# Autodesk Inventor assembly: Manipulator
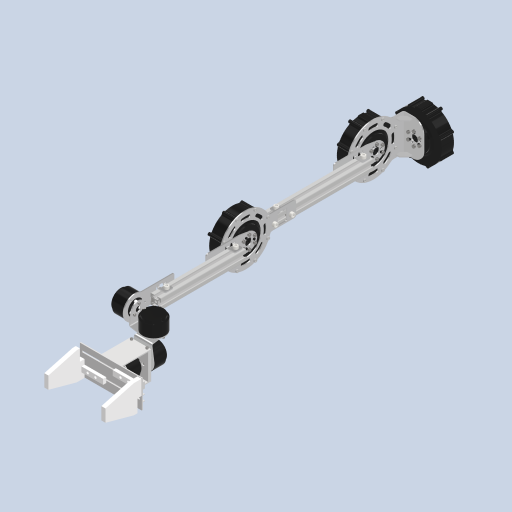
[picture p0: Inventor's stored thumbnail of the model, 512x512]
Saved by Autodesk Inventor 2023 (Build 270158000, 158)
## iProperties
Created: 2024-11-08
Part Number: Manipulator
Document SubType Name: Assembly
Designer: kiyo
Author: kiyo
## Documents named in this file (20)
- D:\GitHub\inventor\syu-si\OfficeRobot\Manipulator\Manipulator.iam
- D:\GitHub\inventor\syu-si\OfficeRobot\ReadyMade\Steadywin\GIM8108-8.iam
- D:\GitHub\inventor\syu-si\OfficeRobot\Manipulator\elbow-pitch-bracket.ipt
- D:\GitHub\inventor\syu-si\OfficeRobot\ReadyMade\Screw\M3_6mm.ipt
- D:\GitHub\inventor\syu-si\OfficeRobot\ReadyMade\Steadywin\GIM3505-8_with-driver.ipt
- D:\GitHub\inventor\syu-si\OfficeRobot\Manipulator\wrist_roll_plate.ipt
- D:\GitHub\inventor\syu-si\OfficeRobot\Manipulator\wrist-pitch-plate.ipt
- D:\GitHub\inventor\syu-si\OfficeRobot\ReadyMade\Screw\M2-5_6mm.ipt
- D:\GitHub\inventor\syu-si\OfficeRobot\ReadyMade\Screw\CBSH3-8.ipt
- D:\GitHub\inventor\syu-si\OfficeRobot\ReadyMade\Screw\FWSJJ-D5-V2_6-T4_5.ipt
- D:\GitHub\inventor\syu-si\OfficeRobot\ReadyMade\Screw\M2-5_10mm.ipt
- D:\GitHub\inventor\syu-si\OfficeRobot\ReadyMade\Screw\HNTU5-5.ipt
- D:\GitHub\inventor\syu-si\OfficeRobot\Manipulator\pitch_plate_20mm.ipt
- D:\GitHub\inventor\syu-si\OfficeRobot\Manipulator\sholder_roll_bracket.ipt
- D:\GitHub\inventor\syu-si\OfficeRobot\ReadyMade\Screw\SCB5-22.ipt
- D:\GitHub\inventor\syu-si\OfficeRobot\ReadyMade\Screw\SCB5-8.ipt
- D:\GitHub\inventor\syu-si\OfficeRobot\Manipulator\Hand_tyokudou.iam
- D:\GitHub\inventor\syu-si\OfficeRobot\Manipulator\wrist-yaw-plate.ipt
- D:\GitHub\inventor\syu-si\OfficeRobot\ReadyMade\Aluminum-frame\NFS5-2020-200-AV10-BV179.ipt
- D:\GitHub\inventor\syu-si\OfficeRobot\ReadyMade\Aluminum-frame\NFS5-2020-165-AV10-BV144.ipt
## Components (91 placed, 19 different names)
1. sholder_roll_bracket:1 — 挿入:350, 挿入:361, 挿入:362, 挿入:363, 挿入:364, 挿入:365, 挿入:366, 挿入:414, 挿入:415
2. wrist-yaw-plate:1 — 挿入:456, 挿入:457, 挿入:458, 挿入:459
3. wrist_roll_plate:2 — 挿入:402, 挿入:403, 挿入:404, 挿入:405, 挿入:406, 挿入:407, 挿入:452
4. Hand_tyokudou:1 [sub-assembly] — 挿入:431, 挿入:434, 挿入:435, 挿入:462, 角度:59, 角度:60
5. pitch_plate_20mm:1 — 挿入:465, 正接:44, メイト:62, 角度:74, 角度:75, 正接:45, メイト:65, メイト:79, 正接:53, 角度:81
6. HNTU5-5:30 — 角度:75
7. SCB5-8:15 — 正接:45, メイト:65
8. elbow-pitch-bracket:1 — 挿入:467, 挿入:468, メイト:81, 正接:55, メイト:85, 正接:57, メイト:87, 正接:58
9. pitch_plate_20mm:2 — 挿入:469, メイト:89, 正接:59, 正接:60, 角度:80, 角度:82
10. wrist-pitch-plate:1 — メイト:70, メイト:71, メイト:72, 正接:46, 正接:47, 正接:48, 正接:49, 角度:76, 角度:77, 角度:78, 正接:50, 正接:51, 挿入:470, 挿入:471
11. NFS5-2020-200-AV10-BV179:1 — 角度:79, メイト:86, メイト:88
12. HNTU5-5:31
13. SCB5-22:9 — メイト:79, 正接:53
14. HNTU5-5:32
15. SCB5-22:10 — メイト:81, 正接:55
16. HNTU5-5:33 — 角度:79, メイト:86
17. SCB5-8:16 — メイト:85, 正接:57
18. HNTU5-5:34 — メイト:88
19. SCB5-8:17 — メイト:87, 正接:58
20. HNTU5-5:35 — 角度:80
21. SCB5-22:11 — メイト:89, 正接:59, 正接:60
22. NFS5-2020-165-AV10-BV144:1
23. M3_6mm:1 — 挿入:337
24. M3_6mm:2 — 挿入:336
25. M3_6mm:3 — 挿入:334
26. M3_6mm:4 — 挿入:338
27. M3_6mm:5 — 挿入:339
28. M3_6mm:6 — 挿入:335
29. M3_6mm:7
30. M3_6mm:8
31. M3_6mm:9
32. M3_6mm:10
33. M3_6mm:11
34. M3_6mm:12
35. M3_6mm:13 — 挿入:361
36. M3_6mm:14 — 挿入:363
37. M3_6mm:15 — 挿入:362
38. M3_6mm:16 — 挿入:364
39. M3_6mm:17 — 挿入:365
40. M3_6mm:18 — 挿入:366
41. CBSH3-8:1 — 挿入:307
42. CBSH3-8:2 — 挿入:308
43. CBSH3-8:3 — 挿入:302
44. CBSH3-8:4 — 挿入:304, 挿入:415
45. CBSH3-8:5 — 挿入:309
46. CBSH3-8:6 — 挿入:303
47. CBSH3-8:7 — 挿入:305
48. CBSH3-8:8 — 挿入:306
49. CBSH3-8:9 — 挿入:332
50. CBSH3-8:10 — 挿入:327, 挿入:468
51. CBSH3-8:11 — 挿入:330
52. CBSH3-8:12 — 挿入:328
53. CBSH3-8:13 — 挿入:329
54. CBSH3-8:14 — 挿入:331
55. CBSH3-8:15 — 挿入:326
56. CBSH3-8:16 — 挿入:333
57. M2-5_6mm:13
58. M2-5_6mm:14
59. M2-5_6mm:15
60. M2-5_10mm:7 — 挿入:402
61. M2-5_10mm:8 — 挿入:403
62. M2-5_10mm:9 — 挿入:404
63. M2-5_10mm:10 — 挿入:430
64. M2-5_10mm:11
65. M2-5_10mm:12
66. M2-5_10mm:13 — 挿入:453, 挿入:456
67. M2-5_10mm:15 — 挿入:454, 挿入:457
68. M2-5_10mm:14 — 挿入:455, 挿入:458
69. FWSJJ-D5-V2_6-T4_5:16 — 挿入:454
70. FWSJJ-D5-V2_6-T4_5:17 — 挿入:453
71. FWSJJ-D5-V2_6-T4_5:18 — 挿入:455
72. FWSJJ-D5-V2_6-T4_5:10 — 挿入:407
73. FWSJJ-D5-V2_6-T4_5:11 — 挿入:405
74. FWSJJ-D5-V2_6-T4_5:12 — 挿入:406
75. FWSJJ-D5-V2_6-T4_5:13 — 挿入:430, 挿入:431
76. FWSJJ-D5-V2_6-T4_5:14 — 挿入:434
77. FWSJJ-D5-V2_6-T4_5:15 — 挿入:435
78. HNTU5-5:22 — 挿入:412, 角度:76
79. SCB5-8:8 — 挿入:412, メイト:72, 正接:49, 正接:50
80. HNTU5-5:23 — 挿入:411, 角度:77
81. SCB5-8:9 — 挿入:411, メイト:71, 正接:48, 正接:51
82. SCB5-22:8 — 挿入:375, メイト:70, 正接:46, 正接:47
83. SCB5-8:7 — 正接:44, メイト:62
84. HNTU5-5:14 — 挿入:375, 角度:78
85. HNTU5-5:21 — 角度:74
86. GIM8108-8:1 [sub-assembly] — 挿入:350, 角度:54, 角度:55, 角度:58
87. GIM8108-8:2 [sub-assembly] — 挿入:302, 挿入:303, 挿入:304, 挿入:305, 挿入:306, 挿入:307, 挿入:308, 挿入:309, 挿入:414, 角度:55, 挿入:465, 角度:81
88. GIM8108-8:3 [sub-assembly] — 挿入:326, 挿入:327, 挿入:328, 挿入:329, 挿入:330, 挿入:331, 挿入:332, 挿入:333, 挿入:334, 挿入:335, 挿入:336, 挿入:337, 挿入:338, 挿入:339, 挿入:467, 挿入:469, 角度:82
89. GIM3505-8_with-driver:9 — 挿入:452, 挿入:470, 挿入:471
90. GIM3505-8_with-driver:8 — 挿入:459
91. GIM3505-8_with-driver:10 — 挿入:462
## Relationships (131: Insert 75, Mate 24, Tangent 18, Angle 14)
- 挿入:302 [Insert] (2 mm): CBSH3-8:3 ↔ GIM8108-8:2
- 挿入:303 [Insert] (2 mm): CBSH3-8:6 ↔ GIM8108-8:2
- 挿入:304 [Insert] (2 mm): CBSH3-8:4 ↔ GIM8108-8:2
- 挿入:305 [Insert] (2 mm): CBSH3-8:7 ↔ GIM8108-8:2
- 挿入:306 [Insert] (2 mm): CBSH3-8:8 ↔ GIM8108-8:2
- 挿入:307 [Insert] (2 mm): CBSH3-8:1 ↔ GIM8108-8:2
- 挿入:308 [Insert] (2 mm): CBSH3-8:2 ↔ GIM8108-8:2
- 挿入:309 [Insert] (2 mm): CBSH3-8:5 ↔ GIM8108-8:2
- 挿入:326 [Insert] (2 mm): CBSH3-8:15 ↔ GIM8108-8:3
- 挿入:327 [Insert] (2 mm): CBSH3-8:10 ↔ GIM8108-8:3
- 挿入:328 [Insert] (2 mm): CBSH3-8:12 ↔ GIM8108-8:3
- 挿入:329 [Insert] (2 mm): CBSH3-8:13 ↔ GIM8108-8:3
- 挿入:330 [Insert] (2 mm): CBSH3-8:11 ↔ GIM8108-8:3
- 挿入:331 [Insert] (2 mm): CBSH3-8:14 ↔ GIM8108-8:3
- 挿入:332 [Insert] (2 mm): CBSH3-8:9 ↔ GIM8108-8:3
- 挿入:333 [Insert] (2 mm): CBSH3-8:16 ↔ GIM8108-8:3
- 挿入:334 [Insert] (2 mm): M3_6mm:3 ↔ GIM8108-8:3
- 挿入:335 [Insert] (2 mm): M3_6mm:6 ↔ GIM8108-8:3
- 挿入:336 [Insert] (2 mm): M3_6mm:2 ↔ GIM8108-8:3
- 挿入:337 [Insert] (2 mm): M3_6mm:1 ↔ GIM8108-8:3
- 挿入:338 [Insert] (2 mm): M3_6mm:4 ↔ GIM8108-8:3
- 挿入:339 [Insert] (2 mm): M3_6mm:5 ↔ GIM8108-8:3
- 挿入:350 [Insert]: sholder_roll_bracket:1 ↔ GIM8108-8:1
- 挿入:361 [Insert]: sholder_roll_bracket:1 ↔ M3_6mm:13
- 挿入:362 [Insert]: sholder_roll_bracket:1 ↔ M3_6mm:15
- 挿入:363 [Insert]: sholder_roll_bracket:1 ↔ M3_6mm:14
- 挿入:364 [Insert]: sholder_roll_bracket:1 ↔ M3_6mm:16
- 挿入:365 [Insert]: sholder_roll_bracket:1 ↔ M3_6mm:17
- 挿入:366 [Insert]: sholder_roll_bracket:1 ↔ M3_6mm:18
- 挿入:375 [Insert] (-0.95 mm): SCB5-22:8 ↔ HNTU5-5:14
- [Insert] (3.2 mm): SCB5-8:7 ↔ HNTU5-5:21
- [Insert]: wrist_roll_plate:2 ↔ M2-5_6mm:13
- [Insert]: wrist_roll_plate:2 ↔ M2-5_6mm:14
- [Insert]: wrist_roll_plate:2 ↔ M2-5_6mm:15
- [Insert]: wrist_roll_plate:2 ↔ GIM3505-8_with-driver:8
- [Insert]: wrist_roll_plate:2 ↔ GIM3505-8_with-driver:8
- 挿入:402 [Insert]: wrist_roll_plate:2 ↔ M2-5_10mm:7
- 挿入:403 [Insert]: wrist_roll_plate:2 ↔ M2-5_10mm:8
- 挿入:404 [Insert]: wrist_roll_plate:2 ↔ M2-5_10mm:9
- 挿入:405 [Insert]: wrist_roll_plate:2 ↔ FWSJJ-D5-V2_6-T4_5:11
- 挿入:406 [Insert]: wrist_roll_plate:2 ↔ FWSJJ-D5-V2_6-T4_5:12
- 挿入:407 [Insert]: wrist_roll_plate:2 ↔ FWSJJ-D5-V2_6-T4_5:10
- 挿入:411 [Insert] (3.5 mm): HNTU5-5:23 ↔ SCB5-8:9
- 挿入:412 [Insert] (3.5 mm): HNTU5-5:22 ↔ SCB5-8:8
- 挿入:414 [Insert]: sholder_roll_bracket:1 ↔ GIM8108-8:2
- 挿入:415 [Insert]: sholder_roll_bracket:1 ↔ CBSH3-8:4
- 挿入:430 [Insert] (2 mm): M2-5_10mm:10 ↔ FWSJJ-D5-V2_6-T4_5:13
- 挿入:431 [Insert]: Hand_tyokudou:1 ↔ FWSJJ-D5-V2_6-T4_5:13
- [Insert] (2 mm): M2-5_10mm:11 ↔ FWSJJ-D5-V2_6-T4_5:14
- [Insert] (2 mm): M2-5_10mm:12 ↔ FWSJJ-D5-V2_6-T4_5:15
- 挿入:434 [Insert]: Hand_tyokudou:1 ↔ FWSJJ-D5-V2_6-T4_5:14
- 挿入:435 [Insert]: Hand_tyokudou:1 ↔ FWSJJ-D5-V2_6-T4_5:15
- 挿入:452 [Insert] (4.5 mm): wrist_roll_plate:2 ↔ GIM3505-8_with-driver:9
- 挿入:453 [Insert] (2 mm): M2-5_10mm:13 ↔ FWSJJ-D5-V2_6-T4_5:17
- 挿入:454 [Insert] (2 mm): M2-5_10mm:15 ↔ FWSJJ-D5-V2_6-T4_5:16
- 挿入:455 [Insert] (2 mm): M2-5_10mm:14 ↔ FWSJJ-D5-V2_6-T4_5:18
- 挿入:456 [Insert]: wrist-yaw-plate:1 ↔ M2-5_10mm:13
- 挿入:457 [Insert]: wrist-yaw-plate:1 ↔ M2-5_10mm:15
- 挿入:458 [Insert]: wrist-yaw-plate:1 ↔ M2-5_10mm:14
- 挿入:459 [Insert] (4.5 mm): wrist-yaw-plate:1 ↔ GIM3505-8_with-driver:8
- [Insert]: wrist-yaw-plate:1 ↔ GIM3505-8_with-driver:10
- [Insert]: wrist-yaw-plate:1 ↔ GIM3505-8_with-driver:10
- 挿入:462 [Insert] (4.5 mm): Hand_tyokudou:1 ↔ GIM3505-8_with-driver:10
- 角度:54 [Angle] (0 deg): GIM8108-8:1
- 角度:55 [Angle] (180 deg): GIM8108-8:1 ↔ GIM8108-8:2
- 角度:58 [Angle] (180 deg): GIM8108-8:1
- 角度:59 [Angle] (0 deg): Hand_tyokudou:1
- 角度:60 [Angle] (0 deg): Hand_tyokudou:1
- 挿入:465 [Insert]: pitch_plate_20mm:1 ↔ GIM8108-8:2
- 正接:44 [Tangent] (0.25 mm): pitch_plate_20mm:1 ↔ SCB5-8:7
- メイト:62 [Mate]: pitch_plate_20mm:1 ↔ SCB5-8:7
- 角度:74 [Angle] (0 deg): pitch_plate_20mm:1 ↔ HNTU5-5:21
- [Insert] (3.2 mm): HNTU5-5:30 ↔ SCB5-8:15
- 角度:75 [Angle] (0 deg): pitch_plate_20mm:1 ↔ HNTU5-5:30
- 正接:45 [Tangent] (0.25 mm): pitch_plate_20mm:1 ↔ SCB5-8:15
- メイト:65 [Mate]: pitch_plate_20mm:1 ↔ SCB5-8:15
- 挿入:467 [Insert]: elbow-pitch-bracket:1 ↔ GIM8108-8:3
- 挿入:468 [Insert]: elbow-pitch-bracket:1 ↔ CBSH3-8:10
- 挿入:469 [Insert]: pitch_plate_20mm:2 ↔ GIM8108-8:3
- メイト:70 [Mate]: wrist-pitch-plate:1 ↔ SCB5-22:8
- メイト:71 [Mate]: wrist-pitch-plate:1 ↔ SCB5-8:9
- メイト:72 [Mate]: wrist-pitch-plate:1 ↔ SCB5-8:8
- 正接:46 [Tangent] (0.25 mm): wrist-pitch-plate:1 ↔ SCB5-22:8
- 正接:47 [Tangent] (7.5 mm): wrist-pitch-plate:1 ↔ SCB5-22:8
- 正接:48 [Tangent] (0.25 mm): wrist-pitch-plate:1 ↔ SCB5-8:9
- 正接:49 [Tangent] (0.25 mm): wrist-pitch-plate:1 ↔ SCB5-8:8
- 角度:76 [Angle] (0 deg): wrist-pitch-plate:1 ↔ HNTU5-5:22
- 角度:77 [Angle] (0 deg): wrist-pitch-plate:1 ↔ HNTU5-5:23
- 角度:78 [Angle] (0 deg): wrist-pitch-plate:1 ↔ HNTU5-5:14
- 正接:50 [Tangent] (7.5 mm): wrist-pitch-plate:1 ↔ SCB5-8:8
- 正接:51 [Tangent] (7.5 mm): wrist-pitch-plate:1 ↔ SCB5-8:9
- 挿入:470 [Insert]: wrist-pitch-plate:1 ↔ GIM3505-8_with-driver:9
- 挿入:471 [Insert]: wrist-pitch-plate:1 ↔ GIM3505-8_with-driver:9
- [Mate]: pitch_plate_20mm:1 ↔ NFS5-2020-200-AV10-BV179:1
- [Mate]: pitch_plate_20mm:1 ↔ NFS5-2020-200-AV10-BV179:1
- [Mate] (1 mm): HNTU5-5:30 ↔ NFS5-2020-200-AV10-BV179:1
- [Mate] (1 mm): NFS5-2020-200-AV10-BV179:1 ↔ HNTU5-5:21
- [Insert] (-0.95 mm): HNTU5-5:31 ↔ SCB5-22:9
- メイト:79 [Mate]: pitch_plate_20mm:1 ↔ SCB5-22:9
- 正接:53 [Tangent] (0.25 mm): pitch_plate_20mm:1 ↔ SCB5-22:9
- [Mate] (1 mm): NFS5-2020-200-AV10-BV179:1 ↔ HNTU5-5:31
- [Tangent] (7.5 mm): NFS5-2020-200-AV10-BV179:1 ↔ SCB5-22:9
- [Insert] (-0.95 mm): HNTU5-5:32 ↔ SCB5-22:10
- メイト:81 [Mate]: elbow-pitch-bracket:1 ↔ SCB5-22:10
- 正接:55 [Tangent] (0.25 mm): elbow-pitch-bracket:1 ↔ SCB5-22:10
- [Mate] (1 mm): NFS5-2020-200-AV10-BV179:1 ↔ HNTU5-5:32
- [Mate]: elbow-pitch-bracket:1 ↔ NFS5-2020-200-AV10-BV179:1
- [Mate]: elbow-pitch-bracket:1 ↔ NFS5-2020-200-AV10-BV179:1
- [Tangent] (18.5 mm): NFS5-2020-200-AV10-BV179:1 ↔ SCB5-22:10
- [Insert] (3.2 mm): HNTU5-5:33 ↔ SCB5-8:16
- メイト:85 [Mate]: elbow-pitch-bracket:1 ↔ SCB5-8:16
- 角度:79 [Angle] (0 deg): NFS5-2020-200-AV10-BV179:1 ↔ HNTU5-5:33
- 正接:57 [Tangent] (0.25 mm): elbow-pitch-bracket:1 ↔ SCB5-8:16
- メイト:86 [Mate] (1 mm): NFS5-2020-200-AV10-BV179:1 ↔ HNTU5-5:33
- [Insert] (3.2 mm): HNTU5-5:34 ↔ SCB5-8:17
- メイト:87 [Mate]: elbow-pitch-bracket:1 ↔ SCB5-8:17
- 正接:58 [Tangent] (0.25 mm): elbow-pitch-bracket:1 ↔ SCB5-8:17
- メイト:88 [Mate] (1 mm): NFS5-2020-200-AV10-BV179:1 ↔ HNTU5-5:34
- [Insert] (-0.95 mm): HNTU5-5:35 ↔ SCB5-22:11
- メイト:89 [Mate]: pitch_plate_20mm:2 ↔ SCB5-22:11
- 正接:59 [Tangent] (0.25 mm): pitch_plate_20mm:2 ↔ SCB5-22:11
- 正接:60 [Tangent] (7.5 mm): pitch_plate_20mm:2 ↔ SCB5-22:11
- 角度:80 [Angle] (0 deg): pitch_plate_20mm:2 ↔ HNTU5-5:35
- [Mate]: pitch_plate_20mm:2 ↔ NFS5-2020-165-AV10-BV144:1
- [Mate]: pitch_plate_20mm:2 ↔ NFS5-2020-165-AV10-BV144:1
- [Tangent] (7.5 mm): SCB5-22:11 ↔ NFS5-2020-165-AV10-BV144:1
- [Mate]: wrist-pitch-plate:1 ↔ NFS5-2020-165-AV10-BV144:1
- [Mate]: wrist-pitch-plate:1 ↔ NFS5-2020-165-AV10-BV144:1
- [Tangent] (18.5 mm): NFS5-2020-165-AV10-BV144:1 ↔ SCB5-22:8
- 角度:81 [Angle] (0 deg): pitch_plate_20mm:1 ↔ GIM8108-8:2
- 角度:82 [Angle] (0 deg): pitch_plate_20mm:2 ↔ GIM8108-8:3
## Named parameters: d492_d466 = 3.2 mm, d516_d512 = 0 mm, d517_d513 = 0 mm, d519_d268 = 0 mm, d520_d269 = 0 mm, d521_d270 = 0 mm, d583_d581 = 2 mm, d584_d581 = 2 mm, d733_d492_d466 = 3.2 mm, d770_d470 = -0.95 mm, d775_d470 = -0.95 mm, d782_d733_d492_d466 = 3.2 mm, d787_d782_d733_d492_d466 = 3.2 mm, d791_d770_d470 = -0.95 mm
